# Autodesk Inventor assembly: Assembly1
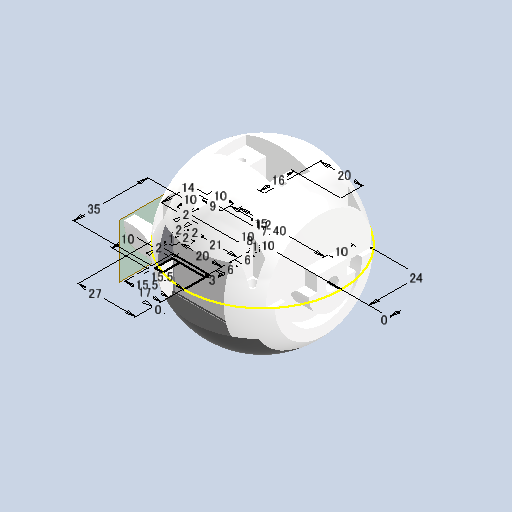
[picture p0: Inventor's stored thumbnail of the model, 512x512]
Saved by Autodesk Inventor 2023 (Build 270158000, 158)
## iProperties
Created: 2022-10-24
Part Number: Assembly1
Document SubType Name: Assembly
Designer: ellie
Author: ellie
## Documents named in this file (8)
- C:\Users\RM206user\Desktop\cansat\tanekonsat2022_runback\machinary\assenbly\Assembly1.iam
- C:\Users\RM206user\Desktop\cansat\tanekonsat2022_runback\machinary\body\body back\back moter middle tire ver\back moter middle tire lemon shape.ipt
- C:\Users\RM206user\Desktop\cansat\tanekonsat2022_runback\machinary\body\body back\back for main connection\body back for main 3.ipt
- C:\Users\RM206user\Desktop\cansat\tanekonsat2022_runback\machinary\body\body front\front moter middle tire\body front moter middle tire 1.ipt
- C:\Users\RM206user\Desktop\cansat\tanekonsat2022_runback\machinary\parts\almi1.ipt
- C:\Users\RM206user\Desktop\cansat\tanekonsat2022_runback\machinary\parts\GNSS1.ipt
- C:\Users\RM206user\Desktop\cansat\tanekonsat2022_runback\machinary\parts\mein1.ipt
- C:\Users\RM206user\Desktop\cansat\tanekonsat2022_runback\machinary\parts\almi2.ipt
## Components (10 placed, 7 different names)
1. body moter middle:1 — メイト:1, メイト:2, メイト:3, メイト:4, メイト:5, メイト:6
2. body moter middle:2 — メイト:1, メイト:2, メイト:3
3. body back:3 — メイト:4, メイト:5, メイト:6
4. base front:1 — メイト:7, メイト:8, メイト:9, メイト:10, メイト:11, メイト:12, メイト:13, メイト:22, メイト:23, メイト:24, メイト:25, メイト:28
5. almi1:1 — メイト:7, メイト:8, メイト:9
6. GNSS1:1 — メイト:10, メイト:11, メイト:23
7. mein1:1 — メイト:12, メイト:13, メイト:22
8. almi2:1 — メイト:26, メイト:27, メイト:28
9. body moter middle:4 — メイト:18, メイト:19, メイト:20, メイト:24, メイト:25, メイト:27
10. body back:5 — メイト:18, メイト:19, メイト:20, メイト:26
## Relationships (23: Mate 23)
- メイト:1 [Mate]: body moter middle:1 ↔ body moter middle:2
- メイト:2 [Mate]: body moter middle:1 ↔ body moter middle:2
- メイト:3 [Mate]: body moter middle:1 ↔ body moter middle:2
- メイト:4 [Mate]: body moter middle:1 ↔ body back:3
- メイト:5 [Mate]: body moter middle:1 ↔ body back:3
- メイト:6 [Mate]: body moter middle:1 ↔ body back:3
- メイト:7 [Mate]: base front:1 ↔ almi1:1
- メイト:8 [Mate]: base front:1 ↔ almi1:1
- メイト:9 [Mate]: base front:1 ↔ almi1:1
- メイト:10 [Mate]: base front:1 ↔ GNSS1:1
- メイト:11 [Mate]: base front:1 ↔ GNSS1:1
- メイト:12 [Mate]: base front:1 ↔ mein1:1
- メイト:13 [Mate]: base front:1 ↔ mein1:1
- メイト:18 [Mate]: body moter middle:4 ↔ body back:5
- メイト:19 [Mate]: body moter middle:4 ↔ body back:5
- メイト:20 [Mate]: body moter middle:4 ↔ body back:5
- メイト:22 [Mate]: base front:1 ↔ mein1:1
- メイト:23 [Mate]: base front:1 ↔ GNSS1:1
- メイト:24 [Mate]: base front:1 ↔ body moter middle:4
- メイト:25 [Mate]: base front:1 ↔ body moter middle:4
- メイト:26 [Mate]: almi2:1 ↔ body back:5
- メイト:27 [Mate]: almi2:1 ↔ body moter middle:4
- メイト:28 [Mate]: base front:1 ↔ almi2:1
